# Autodesk Inventor assembly: HitecMiniServo_HS_82MG
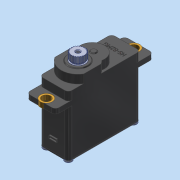
[picture p0: Inventor's stored thumbnail of the model, 180x180]
Saved by Autodesk Inventor 2017 (Build 210142000, 142)
## iProperties
Created: 2018-04-09
Part Number: HitecMiniServo_HS_82MG
Document SubType Name: Assembly
Designer: Derek Wider
Mass: 19.0509 g
Surface Area: 36.9482 cm^2
Volume: 10.1976 cm^3
Author: Derek Wider
## Documents named in this file (5)
- G:\Projects\Submarine\Submarine-project\CAD\common\HitecMiniServo\Assembly\HitecMiniServo_HS_82MG.iam
- G:\Projects\Submarine\Submarine-project\CAD\common\HitecMiniServo\Assembly\ServoBody.ipt
- G:\Projects\Submarine\Submarine-project\CAD\common\HitecMiniServo\Assembly\ScrewHead.ipt
- G:\Projects\Submarine\Submarine-project\CAD\common\HitecMiniServo\Assembly\ServoSpline.ipt
- G:\Projects\Submarine\Submarine-project\CAD\common\HitecMiniServo\Assembly\BrassMountInserts.ipt
## Components (8 placed, 4 different names)
1. ServoBody:1 — Mate:1, Mate:2, Mate:3, Mate:4, Mate:5, Mate:6, Mate:7, Mate:8, Mate:9, Mate:10, Mate:11, Flush:1, Mate:12, Flush:2
2. ScrewHead:1 — Mate:5, Mate:6
3. ServoSpline:1 — Mate:1, Mate:2
4. ScrewHead:2 — Mate:7, Mate:8
5. ScrewHead:3 — Mate:3, Mate:4
6. ScrewHead:4 — Mate:9, Mate:10
7. BrassMountInserts:1 — Mate:12, Flush:2
8. BrassMountInserts:2 — Mate:11, Flush:1
## Relationships (14: Mate 12, Flush 2)
- Mate:1: ServoBody:1 ↔ ServoSpline:1
- Mate:2: ServoBody:1 ↔ ServoSpline:1
- Mate:3: ServoBody:1 ↔ ScrewHead:3
- Mate:4: ServoBody:1 ↔ ScrewHead:3
- Mate:5: ServoBody:1 ↔ ScrewHead:1
- Mate:6: ServoBody:1 ↔ ScrewHead:1
- Mate:7: ServoBody:1 ↔ ScrewHead:2
- Mate:8: ServoBody:1 ↔ ScrewHead:2
- Mate:9: ServoBody:1 ↔ ScrewHead:4
- Mate:10: ServoBody:1 ↔ ScrewHead:4
- Mate:11: ServoBody:1 ↔ BrassMountInserts:2
- Flush:1: ServoBody:1 ↔ BrassMountInserts:2
- Mate:12: ServoBody:1 ↔ BrassMountInserts:1
- Flush:2: ServoBody:1 ↔ BrassMountInserts:1
